# Autodesk Inventor assembly: ミラーマウント２
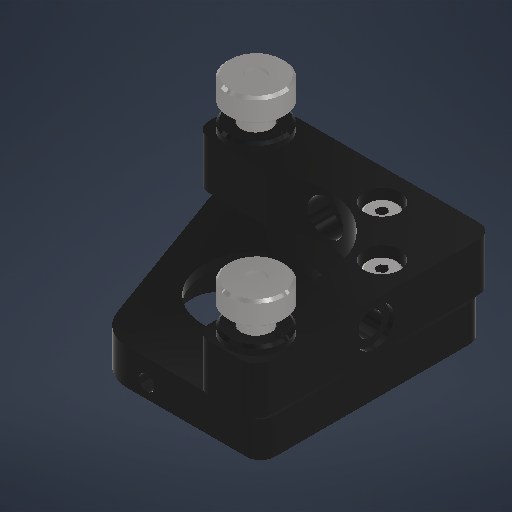
[picture p0: Inventor's stored thumbnail of the model, 512x512]
Saved by Autodesk Inventor 2026 (Build 300175050, 175E)
## iProperties
Created: 2025-07-10
Part Number: ミラーマウント２
Document SubType Name: Assembly
Designer: jin20
Author: jin20
## Documents named in this file (3)
- C:\Users\jin20\Documents\装置CAD\RamanSystem\Optics\ミラーマウント\ミラーマウント.iam
- C:\Users\jin20\Documents\装置CAD\RamanSystem\Optics\ミラーマウント\ミラーマウント_01.ipt
- C:\Users\jin20\Documents\装置CAD\RamanSystem\Optics\ミラーマウント\ミラーマウント_02.ipt
## Components (2 placed, 2 different names)
1. ミラーマウント_01:1 — 挿入:1
2. ミラーマウント_02:1 — 挿入:1
## Relationships (1: Insert 1)
- 挿入:1 [Insert]: ミラーマウント_01:1 ↔ ミラーマウント_02:1
